# Autodesk Inventor assembly: EnsamblajeEslabones
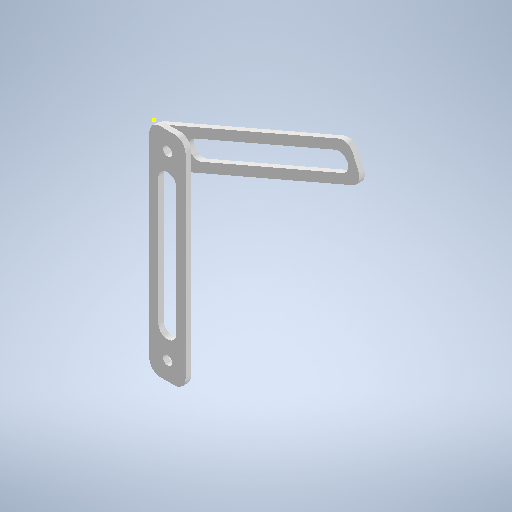
[picture p0: Inventor's stored thumbnail of the model, 512x512]
Saved by Autodesk Inventor 2025 (Build 290162000, 162)
## iProperties
Created: 2024-07-28
Part Number: EnsamblajeEslabones
Document SubType Name: Assembly
Designer: usuario
Author: usuario
## Documents named in this file (3)
- C:\Users\usuario\Desktop\EnsamblajeEslabones.iam
- C:\Users\usuario\Desktop\Eslabon 1.ipt
- C:\Users\usuario\Desktop\Eslabon 2.ipt
## Components (2 placed, 2 different names)
1. Eslabon 1:1 — Coincidencia:1, Coincidencia:2
2. Eslabon 2:1 — Coincidencia:1, Coincidencia:2
## Relationships (2: Mate 2)
- Coincidencia:1 [Mate]: Eslabon 1:1 ↔ Eslabon 2:1
- Coincidencia:2 [Mate]: Eslabon 1:1 ↔ Eslabon 2:1
